# Autodesk Inventor assembly: Bush
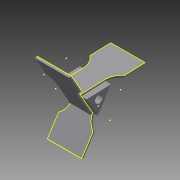
[picture p0: Inventor's stored thumbnail of the model, 180x180]
Saved by Autodesk Inventor 2014 (Build 180170000, 170)
## iProperties
Created: 2014-03-16
Part Number: Bush
Document SubType Name: Assembly
Designer: Pranav
Author: Pranav
## Documents named in this file (3)
- E:\Robotics Autodesk\Old Bush.iam
- E:\Robotics Autodesk\Triangle.ipt
- E:\Robotics Autodesk\Sweep.ipt
## Components (4 placed, 2 different names)
1. Triangle:1 — Mate:1, Mate:2, Mate:3, Mate:4, Mate:5, Mate:6
2. Sweep:1 — Mate:1, Mate:2
3. Sweep:2 — Mate:3, Mate:4
4. Sweep:3 — Mate:5, Mate:6
## Relationships (6: Mate 6)
- Mate:1: Triangle:1 ↔ Sweep:1
- Mate:2: Triangle:1 ↔ Sweep:1
- Mate:3: Triangle:1 ↔ Sweep:2
- Mate:4: Triangle:1 ↔ Sweep:2
- Mate:5: Triangle:1 ↔ Sweep:3
- Mate:6: Triangle:1 ↔ Sweep:3
